# Autodesk Inventor assembly: z motor
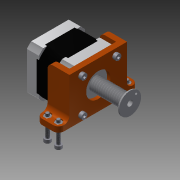
[picture p0: Inventor's stored thumbnail of the model, 180x180]
Saved by Autodesk Inventor 2014 (Build 180170000, 170)
## iProperties
Created: 2013-10-16
Part Number: z motor
Document SubType Name: Assembly
Designer: employee
Author: employee
## Documents named in this file (7)
- \\GRISTLE\speco\GitHub\ConceptFORGE\Wally\z motor.iam
- \\GRISTLE\speco\GitHub\ConceptFORGE\Wally\z motor mount.ipt
- \\GRISTLE\speco\GitHub\ConceptFORGE\Wally\M3x10.ipt
- \\GRISTLE\speco\GitHub\ConceptFORGE\Wally\m3 nut.ipt
- \\GRISTLE\speco\GitHub\ConceptFORGE\Wally\stepper.ipt
- \\GRISTLE\speco\GitHub\ConceptFORGE\Wally\M3x20.ipt
- \\GRISTLE\speco\GitHub\ConceptFORGE\Wally\z pulley.ipt
## Components (15 placed, 6 different names)
1. z motor mount:1 — Insert:1, Insert:2, Insert:3, Insert:4, Angle:1, Angle:2, Angle:3, Angle:4, Insert:5, Insert:6, Insert:7, Insert:8, Insert:9, Angle:5, Insert:10, Insert:11, Insert:12, Insert:13
2. M3x10:1 — Insert:1
3. M3x10:2 — Insert:2
4. M3x10:3 — Insert:3
5. M3x10:4 — Insert:4
6. Hex Nut Metric M3 x 0.5:1 — Angle:4, Insert:5
7. Hex Nut Metric M3 x 0.5:2 — Angle:3, Insert:6
8. Hex Nut Metric M3 x 0.5:3 — Angle:2, Insert:8
9. Hex Nut Metric M3 x 0.5:4 — Angle:1, Insert:7
10. stepper:1 — Insert:9, Angle:5, Insert:14
11. Forged Socket Head Cap Screw - Metric M3x0.5 x 20:1 — Insert:13
12. Forged Socket Head Cap Screw - Metric M3x0.5 x 20:2 — Insert:10
13. Forged Socket Head Cap Screw - Metric M3x0.5 x 20:3 — Insert:11
14. Forged Socket Head Cap Screw - Metric M3x0.5 x 20:4 — Insert:12
15. z pulley:1 — Insert:14
## Relationships (19: Insert 14, Angle 5)
- Insert:1: z motor mount:1 ↔ M3x10:1
- Insert:2: z motor mount:1 ↔ M3x10:2
- Insert:3: z motor mount:1 ↔ M3x10:3
- Insert:4: z motor mount:1 ↔ M3x10:4
- Angle:1 (0 deg): z motor mount:1 ↔ Hex Nut Metric M3 x 0.5:4
- Angle:2 (0 deg): z motor mount:1 ↔ Hex Nut Metric M3 x 0.5:3
- Angle:3 (0 deg): z motor mount:1 ↔ Hex Nut Metric M3 x 0.5:2
- Angle:4 (0 deg): z motor mount:1 ↔ Hex Nut Metric M3 x 0.5:1
- Insert:5: z motor mount:1 ↔ Hex Nut Metric M3 x 0.5:1
- Insert:6: z motor mount:1 ↔ Hex Nut Metric M3 x 0.5:2
- Insert:7: z motor mount:1 ↔ Hex Nut Metric M3 x 0.5:4
- Insert:8: z motor mount:1 ↔ Hex Nut Metric M3 x 0.5:3
- Insert:9: z motor mount:1 ↔ stepper:1
- Angle:5 (0 deg): z motor mount:1 ↔ stepper:1
- Insert:10 (12.5 mm): z motor mount:1 ↔ Forged Socket Head Cap Screw - Metric M3x0.5 x 20:2
- Insert:11 (12.5 mm): z motor mount:1 ↔ Forged Socket Head Cap Screw - Metric M3x0.5 x 20:3
- Insert:12 (12.5 mm): z motor mount:1 ↔ Forged Socket Head Cap Screw - Metric M3x0.5 x 20:4
- Insert:13 (12.5 mm): z motor mount:1 ↔ Forged Socket Head Cap Screw - Metric M3x0.5 x 20:1
- Insert:14: stepper:1 ↔ z pulley:1
